# Autodesk Inventor assembly: b2
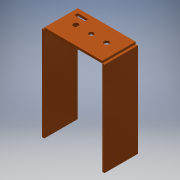
[picture p0: Inventor's stored thumbnail of the model, 180x180]
Saved by Autodesk Inventor 2017 (Build 210142000, 142)
## iProperties
Created: 2015-10-11
Part Number: b2
Document SubType Name: Assembly
Designer: daniel
Author: daniel
## Documents named in this file (3)
- C:\Users\daniel\Documents\GitHub\cardboard-stage-metric\stage\b2.iam
- C:\Users\daniel\Documents\GitHub\cardboard-stage-metric\stage\b1b.ipt
- C:\Users\daniel\Documents\GitHub\cardboard-stage-metric\stage\b2a.ipt
## Components (3 placed, 2 different names)
1. b2a:1 — Flush:3, Mate:3, Mate:4, Mate:5, Mate:6, Mate:7, Flush:4
2. b1b:1 — Flush:3, Mate:3, Mate:6, Mate:7, Flush:5
3. b1b:2 — Mate:4, Mate:5, Flush:4, Flush:5
## Relationships (8: Mate 5, Flush 3)
- Flush:3: b2a:1 ↔ b1b:1
- Mate:3: b2a:1 ↔ b1b:1
- Mate:4: b2a:1 ↔ b1b:2
- Mate:5: b2a:1 ↔ b1b:2
- Mate:6: b2a:1 ↔ b1b:1
- Mate:7: b2a:1 ↔ b1b:1
- Flush:4: b2a:1 ↔ b1b:2
- Flush:5: b1b:1 ↔ b1b:2
